# Autodesk Inventor assembly: AssemblyFull
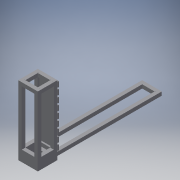
[picture p0: Inventor's stored thumbnail of the model, 180x180]
Saved by Autodesk Inventor 2017 (Build 210142000, 142)
## iProperties
Created: 2019-07-06
Part Number: AssemblyFull
Document SubType Name: Assembly
Designer: Ole Simmering
Author: Ole Simmering
## Documents named in this file (4)
- C:\Users\Ole Simmering\Documents\GitHub\3D_modeling\Guillotine\AssemblyFull.iam
- C:\Users\Ole Simmering\Documents\GitHub\3D_modeling\Guillotine\Assembly.iam
- C:\Users\Ole Simmering\Documents\GitHub\3D_modeling\Guillotine\AssemblyBench.iam
- C:\Users\Ole Simmering\Documents\GitHub\3D_modeling\Guillotine\Bed.iam
## Components (3 placed, 3 different names)
1. Assembly:1 [sub-assembly] — Mate:1, Flush:1, Flush:2
2. AssemblyBench:1 [sub-assembly] — Mate:1, Flush:1, Flush:2, Mate:2, Mate:3, Mate:4
3. Bed:1 [sub-assembly] — Mate:2, Mate:3, Mate:4
## Relationships (6: Mate 4, Flush 2)
- Mate:1: Assembly:1 ↔ AssemblyBench:1
- Flush:1: Assembly:1 ↔ AssemblyBench:1
- Flush:2: Assembly:1 ↔ AssemblyBench:1
- Mate:2: AssemblyBench:1 ↔ Bed:1
- Mate:3: AssemblyBench:1 ↔ Bed:1
- Mate:4: AssemblyBench:1 ↔ Bed:1
